# Autodesk Inventor assembly: Remote Assembly
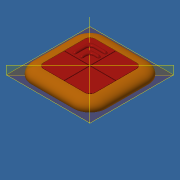
[picture p0: Inventor's stored thumbnail of the model, 180x180]
Saved by Autodesk Inventor 2016 (Build 200138000, 138)
## iProperties
Created: 2015-06-16
Part Number: Remote Assembly
Document SubType Name: Assembly
Designer: Samuel Clay
Author: Samuel Clay
## Documents named in this file (5)
- Z:\turntouch\remote\enclosure\inventor\Remote Assembly.iam
- Z:\turntouch\remote\enclosure\inventor\Remote Top.ipt
- Z:\turntouch\remote\enclosure\inventor\Remote Bottom.ipt
- Z:\turntouch\remote\enclosure\inventor\Remote Buttons.ipt
- Z:\turntouch\remote\enclosure\inventor\Remote Buttons Export.ipt
## Components (4 placed, 4 different names)
1. Remote Top:1 — Flush:1
2. Remote Bottom:1
3. Remote Buttons:1 — Flush:1
4. Remote Buttons Export:1
## Relationships (1: Flush 1)
- Flush:1: Remote Top:1 ↔ Remote Buttons:1
